# Autodesk Inventor assembly: joint4
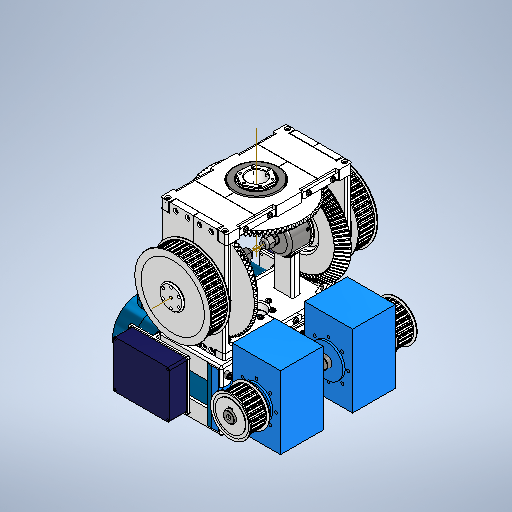
[picture p0: Inventor's stored thumbnail of the model, 512x512]
Saved by Autodesk Inventor 2025.3 (Build 293356030, 356C)
## iProperties
Created: 2025-08-31
Part Number: joint4
Document SubType Name: Assembly
Designer: MSI
Mass: 18202.1 g
Surface Area: 12604.1 cm^2
Volume: 7569.59 cm^3
Density: 2.40463 g/cm^3
Author: MSI
## Documents named in this file (32)
- C:\Users\MSI\Desktop\Project\3. 로봇팔\Robot Arm Model\joint4\joint4.iam
- C:\Users\MSI\Desktop\Project\3. 로봇팔\Robot Arm Model\joint4\encoder.ipt
- C:\Users\MSI\Desktop\Project\3. 로봇팔\Robot Arm Model\joint4\encoder_supporter.ipt
- C:\Users\MSI\Desktop\Project\3. 로봇팔\Robot Arm Model\motor1\motor.iam
- C:\Users\MSI\Desktop\Project\3. 로봇팔\Robot Arm Model\joint4\C-E6704ZZ_Autodesk_Inventor_2024_20250921\C-E6704ZZ.ipt
- C:\Users\MSI\Desktop\Project\3. 로봇팔\Robot Arm Model\joint4\C-E6810ZZ_Autodesk_Inventor_2024_20250921\C-E6810ZZ.ipt
- C:\Users\MSI\Desktop\Project\3. 로봇팔\Robot Arm Model\joint4\NTN_GS81110OuterRings\GS81110Outer Rings.ipt
- C:\Users\MSI\Desktop\Project\3. 로봇팔\Robot Arm Model\joint4\joint4\디자인 액셀러레이터\베벨 기어1.iam
- C:\Users\MSI\Desktop\Project\3. 로봇팔\Robot Arm Model\joint4\joint4\디자인 액셀러레이터\베벨 기어11.ipt
- C:\Users\MSI\Desktop\Project\3. 로봇팔\Robot Arm Model\joint4\joint4_belt_pully2\driven_pulley.iam
- C:\Users\MSI\Desktop\Project\3. 로봇팔\Robot Arm Model\joint4\joint4_belt_pully1\driving_pulley.iam
- C:\Users\MSI\Desktop\Project\3. 로봇팔\Robot Arm Model\joint4\joint4_axis2.ipt
- C:\Users\MSI\Desktop\Project\3. 로봇팔\Robot Arm Model\joint4\joint4_axis3.ipt
- C:\Users\MSI\Desktop\Project\3. 로봇팔\Robot Arm Model\joint4\joint4_pully_cover.ipt
- C:\Users\MSI\Desktop\Project\3. 로봇팔\Robot Arm Model\joint4\joint4_base.ipt
- C:\Users\MSI\Desktop\Project\3. 로봇팔\Robot Arm Model\joint4\joint4_base_carbon.ipt
- C:\Users\MSI\Desktop\Project\3. 로봇팔\Robot Arm Model\joint4\joint4_base_fixture.ipt
- C:\Users\MSI\Desktop\Project\3. 로봇팔\Robot Arm Model\joint4\joint4_base_support_1.ipt
- C:\Users\MSI\Desktop\Project\3. 로봇팔\Robot Arm Model\joint4\joint4_base_support_2.ipt
- C:\Users\MSI\Desktop\Project\3. 로봇팔\Robot Arm Model\joint4\joint4_base_support_fixture.ipt
- C:\Users\MSI\Desktop\Project\3. 로봇팔\Robot Arm Model\joint4\joint4_frame_1.ipt
- C:\Users\MSI\Desktop\Project\3. 로봇팔\Robot Arm Model\joint4\joint4_frame_2.ipt
- C:\Users\MSI\Desktop\Project\3. 로봇팔\Robot Arm Model\joint4\joint4_frame_support_1.ipt
- C:\Users\MSI\Desktop\Project\3. 로봇팔\Robot Arm Model\joint4\joint4_frame_support_2.ipt
- C:\Users\MSI\Desktop\Project\3. 로봇팔\Robot Arm Model\joint4\joint4_frame_support_fixture.ipt
- C:\Users\MSI\Desktop\Project\3. 로봇팔\Robot Arm Model\joint4\joint4_axis2_washer.ipt
- C:\Users\MSI\Desktop\Project\3. 로봇팔\Robot Arm Model\joint4\joint4_axis3_washer.ipt
- C:\Users\MSI\Desktop\Project\3. 로봇팔\Robot Arm Model\joint4\joint4_axis3_washer_2.ipt
- C:\Users\MSI\Documents\Inventor\Content Center Files\R2025\ko-KR\KS B 1023  H (2)\KS B 1023 - A  M 4 x 16 - H(1).ipt
- C:\Users\MSI\Documents\Inventor\Content Center Files\R2025\ko-KR\KS B 1023  H (2)\KS B 1023 - A  M 4 x 25 - H(1).ipt
- C:\Users\MSI\Documents\Inventor\Content Center Files\R2025\ko-KR\KS B 1012  S1\KS B 1012 - A M4(2).ipt
- C:\Users\MSI\Desktop\Project\3. 로봇팔\Robot Arm Model\Robot_Arm_Parameter.xlsx
## Components (176 placed, 30 different names)
1. motor:1 [sub-assembly] — 삽입:8, 삽입:10, 메이트:13, 메이트:14, 각도:1, 메이트:32, 메이트:33, 메이트:34, 메이트:127
2. C-E6704ZZ:1 — 삽입:6, 삽입:31
3. C-E6704ZZ:2 — 삽입:5, 삽입:30
4. C-E6810ZZ:1 — 삽입:32, 삽입:33
5. GS81110Outer Rings:1 — 삽입:13
6. GS81110Outer Rings:2 — 삽입:12, 삽입:34
7. 베벨 기어:1 [sub-assembly] — 메이트:6, 메이트:7, 삽입:11, 삽입:17, 메이트:10, 메이트:45, 메이트:46, 삽입:41, 삽입:42, 삽입:43, 삽입:44, 삽입:45, 삽입:46
8. 베벨 기어1:3 — 메이트:6, 메이트:8, 삽입:9, 메이트:47
9. joint4_axis2:1 — 삽입:9, 메이트:9, 삽입:18
10. joint4_axis2_washer:1 — 삽입:30
11. driven_pulley:1 [sub-assembly] — 삽입:15
12. driving_pulley:1 [sub-assembly] — 삽입:8
13. joint4_pully_cover:1 — 삽입:18, 삽입:15, 삽입:99, 삽입:100, 삽입:101, 삽입:102, 삽입:103, 삽입:104, 삽입:105
14. joint4_axis2:2 — 삽입:11, 삽입:21
15. joint4_axis2_washer:2 — 삽입:31
16. driven_pulley:2 [sub-assembly] — 삽입:16
17. driving_pulley:2 [sub-assembly] — 삽입:10
18. joint4_pully_cover:2 — 삽입:21, 삽입:16, 삽입:106, 삽입:107, 삽입:108, 삽입:109, 삽입:110, 삽입:111, 삽입:112
19. joint4_axis3:1 — 삽입:17, 메이트:10, 삽입:113, 각도:2, 삽입:114, 각도:3, 삽입:115, 각도:4, 삽입:116, 각도:5, 삽입:117, 각도:6, 삽입:118, 각도:7, 삽입:119, 각도:8, 삽입:120, 각도:9, 삽입:121, 각도:10, 삽입:122, 각도:11, 삽입:123, 각도:12, 삽입:124, 각도:13
20. joint4_axis3_washer:1 — 삽입:32, 삽입:14
21. joint4_axis3_washer:2 — 삽입:33
22. joint4_base:1 — 메이트:15, 메이트:16, 메이트:17, 메이트:18, 메이트:19, 메이트:20, 메이트:21, 메이트:22, 메이트:23, 메이트:27, 메이트:29, 메이트:30, 메이트:32, 메이트:33, 메이트:39, 메이트:40, 메이트:41, 메이트:56, 메이트:57, 메이트:58, 삽입:35, 삽입:36, 삽입:40, 삽입:59, 삽입:60, 삽입:61, 삽입:62, 삽입:71, 삽입:72, 삽입:73, 삽입:74
23. joint4_base:2 — 메이트:23, 메이트:24, 메이트:25, 메이트:26, 메이트:28, 메이트:31, 메이트:34, 메이트:42, 메이트:43, 메이트:44, 메이트:45, 메이트:59, 메이트:60, 삽입:37, 삽입:38, 삽입:39, 삽입:63, 삽입:64, 삽입:65, 삽입:66, 삽입:67, 삽입:68, 삽입:69, 삽입:70
24. joint4_base_support_1:1 — 메이트:48, 메이트:49, 메이트:51, 삽입:19, 메이트:56, 메이트:79, 메이트:80, 메이트:81, 메이트:82, 메이트:83, 메이트:84, 메이트:85, 메이트:86, 삽입:51, 삽입:52
25. joint4_base_support_2:1 — 메이트:48, 메이트:49, 메이트:50, 메이트:57, 메이트:58, 삽입:53, 삽입:54
26. joint4_base_carbon:5 — 메이트:79, 메이트:80
27. joint4_base_carbon:6 — 메이트:81, 메이트:82
28. joint4_base_carbon:7 — 메이트:83, 메이트:84
29. joint4_base_carbon:8 — 메이트:85, 메이트:86
30. joint4_base_support_fixture:1 — 메이트:50, 메이트:51, 삽입:75, 삽입:76
31. joint4_base_support_1:2 — 메이트:60, 삽입:55, 삽입:56
32. joint4_base_support_2:2 — 삽입:20, 메이트:59, 메이트:87, 메이트:88, 메이트:89, 메이트:90, 메이트:91, 메이트:92, 메이트:93, 메이트:94, 삽입:57, 삽입:58
33. joint4_base_carbon:9 — 메이트:87, 메이트:88
34. joint4_base_carbon:10 — 메이트:89, 메이트:90
35. joint4_base_carbon:11 — 메이트:91, 메이트:92
36. joint4_base_carbon:12 — 메이트:93, 메이트:94
37. joint4_base_support_fixture:2 — 삽입:77, 삽입:78
38. joint4_base_carbon:1 — 메이트:15, 메이트:16, 메이트:24
39. joint4_base_carbon:2 — 메이트:17, 메이트:18
40. joint4_base_carbon:3 — 메이트:19, 메이트:20
41. joint4_base_carbon:4 — 메이트:21, 메이트:22, 메이트:25
42. joint4_base_fixture:1 — 메이트:29, 메이트:30, 메이트:31, 삽입:49, 삽입:50
43. joint4_base_fixture:2 — 메이트:26, 메이트:27, 메이트:28, 삽입:47, 삽입:48
44. encoder_supporter:1 — 삽입:4, 메이트:42, 메이트:43, 메이트:44
45. encoder_supporter:2 — 삽입:7, 메이트:39, 메이트:40, 메이트:41
46. encoder:1 — 삽입:7, 메이트:47
47. encoder:2 — 삽입:4, 메이트:46
48. C-E6704ZZ:3 — 삽입:19
49. C-E6704ZZ:4 — 삽입:20
50. joint4_frame_1:1 — 메이트:63, 메이트:64, 삽입:27, 삽입:29, 메이트:75, 메이트:76, 메이트:78, 삽입:91, 삽입:92, 메이트:134
51. joint4_base_carbon:13 — 메이트:95, 메이트:96
52. joint4_base_carbon:14 — 메이트:97, 메이트:98
53. joint4_base_carbon:15 — 메이트:99, 메이트:100
54. joint4_base_carbon:16 — 메이트:101, 메이트:102
55. joint4_frame_1:2 — 메이트:61, 메이트:62, 삽입:23, 삽입:24, 메이트:73, 메이트:74, 메이트:77, 삽입:97, 삽입:98
56. joint4_base_carbon:17 — 메이트:103, 메이트:104
57. joint4_base_carbon:18 — 메이트:105, 메이트:106
58. joint4_base_carbon:19 — 메이트:107, 메이트:108
59. joint4_base_carbon:20 — 메이트:109, 메이트:110
60. joint4_frame_2:1 — 메이트:61, 메이트:62, 삽입:22, 메이트:64, 삽입:28, 메이트:7, 삽입:12, 삽입:13, 삽입:14, 메이트:77, 메이트:78, 메이트:95, 메이트:96, 메이트:97, 메이트:98, 메이트:99, 메이트:101, 메이트:103, 메이트:105, 메이트:107, 메이트:108, 메이트:109, 메이트:110, 메이트:133
61. joint4_frame_2:2 — 메이트:129, 메이트:130, 메이트:131, 메이트:132, 메이트:133, 메이트:134, 삽입:25, 메이트:63, 메이트:102, 메이트:100, 메이트:104, 메이트:106, 삽입:26
62. joint4_base_carbon:29 — 메이트:129, 메이트:130
63. joint4_base_carbon:30 — 메이트:131, 메이트:132
64. joint4_base_fixture:3 — 삽입:22, 삽입:23, 삽입:85, 삽입:86
65. joint4_base_fixture:4 — 삽입:24, 삽입:81, 삽입:82, 삽입:26
66. joint4_base_fixture:6 — 삽입:27, 삽입:79, 삽입:80, 삽입:25
67. joint4_base_fixture:5 — 삽입:28, 삽입:29, 삽입:83, 삽입:84
68. joint4_frame_support_1:1 — 메이트:65, 메이트:66, 메이트:67, 메이트:73, 삽입:6, 메이트:8, 메이트:9, 삽입:93, 삽입:94
69. joint4_base_carbon:25 — 메이트:119, 메이트:120
70. joint4_base_carbon:26 — 메이트:121, 메이트:122
71. joint4_base_carbon:27 — 메이트:123, 메이트:124
72. joint4_base_carbon:28 — 메이트:125, 메이트:126
73. joint4_frame_support_2:1 — 메이트:65, 메이트:66, 메이트:68, 메이트:74, 메이트:119, 메이트:120, 메이트:121, 메이트:122, 메이트:123, 메이트:124, 메이트:125, 메이트:126, 삽입:95, 삽입:96
74. joint4_frame_support_fixture:1 — 메이트:67, 메이트:68, 삽입:127, 삽입:128
75. joint4_frame_support_1:2 — 메이트:75, 메이트:111, 메이트:112, 메이트:113, 메이트:114, 메이트:115, 메이트:116, 메이트:117, 메이트:118, 삽입:87, 삽입:88
76. joint4_base_carbon:21 — 메이트:111, 메이트:112
77. joint4_base_carbon:22 — 메이트:113, 메이트:114
78. joint4_base_carbon:23 — 메이트:115, 메이트:116
79. joint4_base_carbon:24 — 메이트:117, 메이트:118
80. joint4_frame_support_2:2 — 메이트:76, 삽입:5, 삽입:89, 삽입:90
81. joint4_frame_support_fixture:2 — 삽입:125, 삽입:126
82. joint4_axis3_washer_2:1 — 삽입:34
83. KS B 1023 H - 미터 A  M 4 x 16 - H:1 — 삽입:47
84. KS B 1023 H - 미터 A  M 4 x 25 - H:1 — 삽입:36
85. KS B 1012 스타일 1 - 미터 A M4:1 — 삽입:113, 각도:2
86. KS B 1023 H - 미터 A  M 4 x 25 - H:2 — 삽입:35
87. KS B 1023 H - 미터 A  M 4 x 25 - H:3 — 삽입:40
88. KS B 1023 H - 미터 A  M 4 x 25 - H:4 — 삽입:38
89. KS B 1023 H - 미터 A  M 4 x 25 - H:5 — 삽입:39
90. KS B 1023 H - 미터 A  M 4 x 25 - H:6 — 삽입:37
91. KS B 1023 H - 미터 A  M 4 x 25 - H:7 — 삽입:41
92. KS B 1023 H - 미터 A  M 4 x 25 - H:8 — 삽입:46
93. KS B 1023 H - 미터 A  M 4 x 25 - H:9 — 삽입:45
94. KS B 1023 H - 미터 A  M 4 x 25 - H:10 — 삽입:43
95. KS B 1023 H - 미터 A  M 4 x 25 - H:11 — 삽입:44
96. KS B 1023 H - 미터 A  M 4 x 25 - H:12 — 삽입:42
97. KS B 1023 H - 미터 A  M 4 x 16 - H:2 — 삽입:48
98. KS B 1023 H - 미터 A  M 4 x 16 - H:3 — 삽입:49
99. KS B 1023 H - 미터 A  M 4 x 16 - H:4 — 삽입:50
100. KS B 1023 H - 미터 A  M 4 x 16 - H:5 — 삽입:52
101. KS B 1023 H - 미터 A  M 4 x 16 - H:6 — 삽입:53
102. KS B 1023 H - 미터 A  M 4 x 16 - H:7 — 삽입:54
103. KS B 1023 H - 미터 A  M 4 x 16 - H:8 — 삽입:51
104. KS B 1023 H - 미터 A  M 4 x 16 - H:9 — 삽입:56
105. KS B 1023 H - 미터 A  M 4 x 16 - H:10 — 삽입:57
106. KS B 1023 H - 미터 A  M 4 x 16 - H:11 — 삽입:55
107. KS B 1023 H - 미터 A  M 4 x 16 - H:12 — 삽입:58
108. KS B 1023 H - 미터 A  M 4 x 16 - H:13 — 삽입:60
109. KS B 1023 H - 미터 A  M 4 x 16 - H:14 — 삽입:59
110. KS B 1023 H - 미터 A  M 4 x 16 - H:15 — 삽입:62
111. KS B 1023 H - 미터 A  M 4 x 16 - H:16 — 삽입:61
112. KS B 1023 H - 미터 A  M 4 x 16 - H:17 — 삽입:64
113. KS B 1023 H - 미터 A  M 4 x 16 - H:18 — 삽입:63
114. KS B 1023 H - 미터 A  M 4 x 16 - H:19 — 삽입:65
115. KS B 1023 H - 미터 A  M 4 x 16 - H:20 — 삽입:66
116. KS B 1023 H - 미터 A  M 4 x 16 - H:21 — 삽입:72
117. KS B 1023 H - 미터 A  M 4 x 16 - H:22 — 삽입:71
118. KS B 1023 H - 미터 A  M 4 x 16 - H:23 — 삽입:74
119. KS B 1023 H - 미터 A  M 4 x 16 - H:24 — 삽입:73
120. KS B 1023 H - 미터 A  M 4 x 16 - H:25 — 삽입:67
121. KS B 1023 H - 미터 A  M 4 x 16 - H:26 — 삽입:68
122. KS B 1023 H - 미터 A  M 4 x 16 - H:27 — 삽입:70
123. KS B 1023 H - 미터 A  M 4 x 16 - H:28 — 삽입:69
124. KS B 1023 H - 미터 A  M 4 x 16 - H:29 — 삽입:76
125. KS B 1023 H - 미터 A  M 4 x 16 - H:30 — 삽입:75
126. KS B 1023 H - 미터 A  M 4 x 16 - H:31 — 삽입:78
127. KS B 1023 H - 미터 A  M 4 x 16 - H:32 — 삽입:77
128. KS B 1023 H - 미터 A  M 4 x 16 - H:33 — 삽입:88
129. KS B 1023 H - 미터 A  M 4 x 16 - H:34 — 삽입:89
130. KS B 1023 H - 미터 A  M 4 x 16 - H:35 — 삽입:90
131. KS B 1023 H - 미터 A  M 4 x 16 - H:36 — 삽입:87
132. KS B 1023 H - 미터 A  M 4 x 16 - H:37 — 삽입:94
133. KS B 1023 H - 미터 A  M 4 x 16 - H:38 — 삽입:95
134. KS B 1023 H - 미터 A  M 4 x 16 - H:39 — 삽입:93
135. KS B 1023 H - 미터 A  M 4 x 16 - H:40 — 삽입:96
136. KS B 1023 H - 미터 A  M 4 x 16 - H:41 — 삽입:91
137. KS B 1023 H - 미터 A  M 4 x 16 - H:42 — 삽입:92
138. KS B 1023 H - 미터 A  M 4 x 16 - H:43 — 삽입:98
139. KS B 1023 H - 미터 A  M 4 x 16 - H:44 — 삽입:97
140. KS B 1023 H - 미터 A  M 4 x 16 - H:45 — 삽입:79
141. KS B 1023 H - 미터 A  M 4 x 16 - H:46 — 삽입:80
142. KS B 1023 H - 미터 A  M 4 x 16 - H:47 — 삽입:83
143. KS B 1023 H - 미터 A  M 4 x 16 - H:48 — 삽입:84
144. KS B 1023 H - 미터 A  M 4 x 16 - H:49 — 삽입:81
145. KS B 1023 H - 미터 A  M 4 x 16 - H:50 — 삽입:82
146. KS B 1023 H - 미터 A  M 4 x 16 - H:51 — 삽입:85
147. KS B 1023 H - 미터 A  M 4 x 16 - H:52 — 삽입:86
148. KS B 1023 H - 미터 A  M 4 x 16 - H:53 — 삽입:100
149. KS B 1023 H - 미터 A  M 4 x 16 - H:54 — 삽입:101
150. KS B 1023 H - 미터 A  M 4 x 16 - H:55 — 삽입:102
151. KS B 1023 H - 미터 A  M 4 x 16 - H:56 — 삽입:103
152. KS B 1023 H - 미터 A  M 4 x 16 - H:57 — 삽입:104
153. KS B 1023 H - 미터 A  M 4 x 16 - H:58 — 삽입:105
154. KS B 1023 H - 미터 A  M 4 x 16 - H:59 — 삽입:99
155. KS B 1023 H - 미터 A  M 4 x 16 - H:60 — 삽입:107
156. KS B 1023 H - 미터 A  M 4 x 16 - H:61 — 삽입:108
157. KS B 1023 H - 미터 A  M 4 x 16 - H:62 — 삽입:109
158. KS B 1023 H - 미터 A  M 4 x 16 - H:63 — 삽입:110
159. KS B 1023 H - 미터 A  M 4 x 16 - H:64 — 삽입:111
160. KS B 1023 H - 미터 A  M 4 x 16 - H:65 — 삽입:112
161. KS B 1023 H - 미터 A  M 4 x 16 - H:66 — 삽입:106
162. KS B 1012 스타일 1 - 미터 A M4:2 — 삽입:114, 각도:3
163. KS B 1012 스타일 1 - 미터 A M4:3 — 삽입:115, 각도:4
164. KS B 1012 스타일 1 - 미터 A M4:4 — 삽입:116, 각도:5
165. KS B 1012 스타일 1 - 미터 A M4:5 — 삽입:117, 각도:6
166. KS B 1012 스타일 1 - 미터 A M4:6 — 삽입:118, 각도:7
167. KS B 1012 스타일 1 - 미터 A M4:7 — 삽입:120, 각도:9
168. KS B 1012 스타일 1 - 미터 A M4:8 — 삽입:119, 각도:8
169. KS B 1012 스타일 1 - 미터 A M4:9 — 삽입:121, 각도:10
170. KS B 1012 스타일 1 - 미터 A M4:10 — 삽입:122, 각도:11
171. KS B 1012 스타일 1 - 미터 A M4:11 — 삽입:123, 각도:12
172. KS B 1012 스타일 1 - 미터 A M4:12 — 삽입:124, 각도:13
173. KS B 1023 H - 미터 A  M 4 x 16 - H:67 — 삽입:125
174. KS B 1023 H - 미터 A  M 4 x 16 - H:68 — 삽입:126
175. KS B 1023 H - 미터 A  M 4 x 16 - H:69 — 삽입:127
176. KS B 1023 H - 미터 A  M 4 x 16 - H:70 — 삽입:128
## Relationships (260: Insert 125, Mate 122, Angle 13)
- 삽입:4 [Insert]: encoder_supporter:1 ↔ encoder:2
- 삽입:5 [Insert]: C-E6704ZZ:2 ↔ joint4_frame_support_2:2
- 삽입:6 [Insert]: C-E6704ZZ:1 ↔ joint4_frame_support_1:1
- 메이트:6 [Mate]: 베벨 기어:1 ↔ 베벨 기어1:3
- 삽입:7 [Insert]: encoder_supporter:2 ↔ encoder:1
- 메이트:7 [Mate]: 베벨 기어:1 ↔ joint4_frame_2:1
- 메이트:8 [Mate]: 베벨 기어1:3 ↔ joint4_frame_support_1:1
- 삽입:8 [Insert]: motor:1 ↔ driving_pulley:1
- 삽입:9 [Insert]: 베벨 기어1:3 ↔ joint4_axis2:1
- 삽입:10 [Insert]: motor:1 ↔ driving_pulley:2
- 삽입:11 [Insert]: 베벨 기어:1 ↔ joint4_axis2:2
- 삽입:12 [Insert]: GS81110Outer Rings:2 ↔ joint4_frame_2:1
- 삽입:13 [Insert]: GS81110Outer Rings:1 ↔ joint4_frame_2:1
- 삽입:14 [Insert] (0.25 mm): joint4_axis3_washer:1 ↔ joint4_frame_2:1
- 메이트:9 [Mate]: joint4_axis2:1 ↔ joint4_frame_support_1:1
- 삽입:15 [Insert]: driven_pulley:1 ↔ joint4_pully_cover:1
- 삽입:16 [Insert]: driven_pulley:2 ↔ joint4_pully_cover:2
- 삽입:17 [Insert]: 베벨 기어:1 ↔ joint4_axis3:1
- 메이트:10 [Mate]: 베벨 기어:1 ↔ joint4_axis3:1
- 삽입:18 [Insert] (0.5 mm): joint4_axis2:1 ↔ joint4_pully_cover:1
- 메이트:13 [Mate]: motor:1
- 메이트:14 [Mate]: motor:1
- 각도:1 [Angle] (0 deg): motor:1
- 메이트:15 [Mate]: joint4_base:1 ↔ joint4_base_carbon:1
- 메이트:16 [Mate]: joint4_base:1 ↔ joint4_base_carbon:1
- 메이트:17 [Mate]: joint4_base:1 ↔ joint4_base_carbon:2
- 메이트:18 [Mate]: joint4_base:1 ↔ joint4_base_carbon:2
- 메이트:19 [Mate]: joint4_base:1 ↔ joint4_base_carbon:3
- 메이트:20 [Mate]: joint4_base:1 ↔ joint4_base_carbon:3
- 메이트:21 [Mate]: joint4_base:1 ↔ joint4_base_carbon:4
- 메이트:22 [Mate]: joint4_base:1 ↔ joint4_base_carbon:4
- 메이트:23 [Mate]: joint4_base:1 ↔ joint4_base:2
- 메이트:24 [Mate]: joint4_base:2 ↔ joint4_base_carbon:1
- 메이트:25 [Mate]: joint4_base:2 ↔ joint4_base_carbon:4
- 메이트:26 [Mate]: joint4_base:2 ↔ joint4_base_fixture:2
- 메이트:27 [Mate]: joint4_base:1 ↔ joint4_base_fixture:2
- 메이트:28 [Mate]: joint4_base:2 ↔ joint4_base_fixture:2
- 메이트:29 [Mate]: joint4_base:1 ↔ joint4_base_fixture:1
- 메이트:30 [Mate]: joint4_base:1 ↔ joint4_base_fixture:1
- 메이트:31 [Mate]: joint4_base:2 ↔ joint4_base_fixture:1
- 메이트:32 [Mate]: motor:1 ↔ joint4_base:1
- 메이트:33 [Mate]: motor:1 ↔ joint4_base:1
- 메이트:34 [Mate]: motor:1 ↔ joint4_base:2
- 메이트:39 [Mate]: joint4_base:1 ↔ encoder_supporter:2
- 메이트:40 [Mate]: joint4_base:1 ↔ encoder_supporter:2
- 메이트:41 [Mate]: joint4_base:1 ↔ encoder_supporter:2
- 메이트:42 [Mate]: joint4_base:2 ↔ encoder_supporter:1
- 메이트:43 [Mate]: joint4_base:2 ↔ encoder_supporter:1
- 메이트:44 [Mate]: joint4_base:2 ↔ encoder_supporter:1
- 메이트:45 [Mate]: 베벨 기어:1 ↔ joint4_base:2
- 메이트:46 [Mate]: 베벨 기어:1 ↔ encoder:2
- 메이트:47 [Mate]: 베벨 기어1:3 ↔ encoder:1
- 메이트:48 [Mate]: joint4_base_support_1:1 ↔ joint4_base_support_2:1
- 메이트:49 [Mate]: joint4_base_support_1:1 ↔ joint4_base_support_2:1
- 메이트:50 [Mate]: joint4_base_support_2:1 ↔ joint4_base_support_fixture:1
- 메이트:51 [Mate]: joint4_base_support_1:1 ↔ joint4_base_support_fixture:1
- [Mate]: joint4_base_support_1:2 ↔ joint4_base_support_2:2
- [Mate]: joint4_base_support_1:2 ↔ joint4_base_support_2:2
- [Mate]: joint4_base_support_2:2 ↔ joint4_base_support_fixture:2
- [Mate]: joint4_base_support_1:2 ↔ joint4_base_support_fixture:2
- 삽입:19 [Insert]: joint4_base_support_1:1 ↔ C-E6704ZZ:3
- 메이트:56 [Mate]: joint4_base:1 ↔ joint4_base_support_1:1
- 메이트:57 [Mate]: joint4_base:1 ↔ joint4_base_support_2:1
- 메이트:58 [Mate]: joint4_base:1 ↔ joint4_base_support_2:1
- 삽입:20 [Insert]: joint4_base_support_2:2 ↔ C-E6704ZZ:4
- 메이트:59 [Mate]: joint4_base:2 ↔ joint4_base_support_2:2
- 메이트:60 [Mate]: joint4_base:2 ↔ joint4_base_support_1:2
- 삽입:21 [Insert] (0.5 mm): joint4_axis2:2 ↔ joint4_pully_cover:2
- 메이트:61 [Mate]: joint4_frame_1:2 ↔ joint4_frame_2:1
- 메이트:62 [Mate]: joint4_frame_1:2 ↔ joint4_frame_2:1
- 삽입:22 [Insert]: joint4_frame_2:1 ↔ joint4_base_fixture:3
- 삽입:23 [Insert]: joint4_frame_1:2 ↔ joint4_base_fixture:3
- 삽입:24 [Insert]: joint4_frame_1:2 ↔ joint4_base_fixture:4
- 삽입:25 [Insert]: joint4_frame_2:2 ↔ joint4_base_fixture:6
- 메이트:63 [Mate]: joint4_frame_1:1 ↔ joint4_frame_2:2
- 메이트:64 [Mate]: joint4_frame_1:1 ↔ joint4_frame_2:1
- 삽입:26 [Insert]: joint4_frame_2:2 ↔ joint4_base_fixture:4
- 삽입:27 [Insert]: joint4_frame_1:1 ↔ joint4_base_fixture:6
- 삽입:28 [Insert]: joint4_frame_2:1 ↔ joint4_base_fixture:5
- 삽입:29 [Insert]: joint4_frame_1:1 ↔ joint4_base_fixture:5
- 메이트:65 [Mate]: joint4_frame_support_1:1 ↔ joint4_frame_support_2:1
- 메이트:66 [Mate]: joint4_frame_support_1:1 ↔ joint4_frame_support_2:1
- 메이트:67 [Mate]: joint4_frame_support_1:1 ↔ joint4_frame_support_fixture:1
- 메이트:68 [Mate]: joint4_frame_support_2:1 ↔ joint4_frame_support_fixture:1
- [Mate]: joint4_frame_support_1:2 ↔ joint4_frame_support_2:2
- [Mate]: joint4_frame_support_1:2 ↔ joint4_frame_support_2:2
- [Mate]: joint4_frame_support_1:2 ↔ joint4_frame_support_fixture:2
- [Mate]: joint4_frame_support_2:2 ↔ joint4_frame_support_fixture:2
- 메이트:73 [Mate]: joint4_frame_1:2 ↔ joint4_frame_support_1:1
- 메이트:74 [Mate]: joint4_frame_1:2 ↔ joint4_frame_support_2:1
- 메이트:75 [Mate]: joint4_frame_1:1 ↔ joint4_frame_support_1:2
- 메이트:76 [Mate]: joint4_frame_1:1 ↔ joint4_frame_support_2:2
- 메이트:77 [Mate] (0.5 mm): joint4_frame_1:2 ↔ joint4_frame_2:1
- 메이트:78 [Mate] (0.5 mm): joint4_frame_1:1 ↔ joint4_frame_2:1
- 메이트:79 [Mate] (0.25 mm): joint4_base_support_1:1 ↔ joint4_base_carbon:5
- 메이트:80 [Mate]: joint4_base_support_1:1 ↔ joint4_base_carbon:5
- 메이트:81 [Mate] (0.25 mm): joint4_base_support_1:1 ↔ joint4_base_carbon:6
- 메이트:82 [Mate]: joint4_base_support_1:1 ↔ joint4_base_carbon:6
- 메이트:83 [Mate] (0.25 mm): joint4_base_support_1:1 ↔ joint4_base_carbon:7
- 메이트:84 [Mate]: joint4_base_support_1:1 ↔ joint4_base_carbon:7
- 메이트:85 [Mate] (0.25 mm): joint4_base_support_1:1 ↔ joint4_base_carbon:8
- 메이트:86 [Mate]: joint4_base_support_1:1 ↔ joint4_base_carbon:8
- 메이트:87 [Mate] (0.25 mm): joint4_base_support_2:2 ↔ joint4_base_carbon:9
- 메이트:88 [Mate]: joint4_base_support_2:2 ↔ joint4_base_carbon:9
- 메이트:89 [Mate] (0.25 mm): joint4_base_support_2:2 ↔ joint4_base_carbon:10
- 메이트:90 [Mate]: joint4_base_support_2:2 ↔ joint4_base_carbon:10
- 메이트:91 [Mate] (0.25 mm): joint4_base_support_2:2 ↔ joint4_base_carbon:11
- 메이트:92 [Mate]: joint4_base_support_2:2 ↔ joint4_base_carbon:11
- 메이트:93 [Mate] (0.25 mm): joint4_base_support_2:2 ↔ joint4_base_carbon:12
- 메이트:94 [Mate]: joint4_base_support_2:2 ↔ joint4_base_carbon:12
- 메이트:95 [Mate] (0.25 mm): joint4_base_carbon:13 ↔ joint4_frame_2:1
- 메이트:96 [Mate]: joint4_base_carbon:13 ↔ joint4_frame_2:1
- 메이트:97 [Mate] (0.25 mm): joint4_base_carbon:14 ↔ joint4_frame_2:1
- 메이트:98 [Mate]: joint4_base_carbon:14 ↔ joint4_frame_2:1
- 메이트:99 [Mate] (0.25 mm): joint4_base_carbon:15 ↔ joint4_frame_2:1
- 메이트:100 [Mate]: joint4_base_carbon:15 ↔ joint4_frame_2:2
- 메이트:101 [Mate] (0.25 mm): joint4_base_carbon:16 ↔ joint4_frame_2:1
- 메이트:102 [Mate]: joint4_base_carbon:16 ↔ joint4_frame_2:2
- 메이트:103 [Mate] (0.25 mm): joint4_base_carbon:17 ↔ joint4_frame_2:1
- 메이트:104 [Mate]: joint4_base_carbon:17 ↔ joint4_frame_2:2
- 메이트:105 [Mate] (0.25 mm): joint4_base_carbon:18 ↔ joint4_frame_2:1
- 메이트:106 [Mate]: joint4_base_carbon:18 ↔ joint4_frame_2:2
- 메이트:107 [Mate] (0.25 mm): joint4_base_carbon:19 ↔ joint4_frame_2:1
- 메이트:108 [Mate]: joint4_base_carbon:19 ↔ joint4_frame_2:1
- 메이트:109 [Mate] (0.25 mm): joint4_base_carbon:20 ↔ joint4_frame_2:1
- 메이트:110 [Mate]: joint4_base_carbon:20 ↔ joint4_frame_2:1
- 메이트:111 [Mate] (0.25 mm): joint4_frame_support_1:2 ↔ joint4_base_carbon:21
- 메이트:112 [Mate]: joint4_frame_support_1:2 ↔ joint4_base_carbon:21
- 메이트:113 [Mate] (0.25 mm): joint4_frame_support_1:2 ↔ joint4_base_carbon:22
- 메이트:114 [Mate]: joint4_frame_support_1:2 ↔ joint4_base_carbon:22
- 메이트:115 [Mate] (0.25 mm): joint4_frame_support_1:2 ↔ joint4_base_carbon:23
- 메이트:116 [Mate]: joint4_frame_support_1:2 ↔ joint4_base_carbon:23
- 메이트:117 [Mate] (0.25 mm): joint4_frame_support_1:2 ↔ joint4_base_carbon:24
- 메이트:118 [Mate]: joint4_frame_support_1:2 ↔ joint4_base_carbon:24
- 메이트:119 [Mate] (0.25 mm): joint4_base_carbon:25 ↔ joint4_frame_support_2:1
- 메이트:120 [Mate]: joint4_base_carbon:25 ↔ joint4_frame_support_2:1
- 메이트:121 [Mate] (0.25 mm): joint4_base_carbon:26 ↔ joint4_frame_support_2:1
- 메이트:122 [Mate]: joint4_base_carbon:26 ↔ joint4_frame_support_2:1
- 메이트:123 [Mate] (0.25 mm): joint4_base_carbon:27 ↔ joint4_frame_support_2:1
- 메이트:124 [Mate]: joint4_base_carbon:27 ↔ joint4_frame_support_2:1
- 메이트:125 [Mate] (0.25 mm): joint4_base_carbon:28 ↔ joint4_frame_support_2:1
- 메이트:126 [Mate]: joint4_base_carbon:28 ↔ joint4_frame_support_2:1
- 삽입:30 [Insert] (0.5 mm): C-E6704ZZ:2 ↔ joint4_axis2_washer:1
- 삽입:31 [Insert] (0.5 mm): C-E6704ZZ:1 ↔ joint4_axis2_washer:2
- 삽입:32 [Insert] (0.25 mm): C-E6810ZZ:1 ↔ joint4_axis3_washer:1
- 삽입:33 [Insert] (0.25 mm): C-E6810ZZ:1 ↔ joint4_axis3_washer:2
- 삽입:34 [Insert] (0.5 mm): GS81110Outer Rings:2 ↔ joint4_axis3_washer_2:1
- 삽입:35 [Insert]: joint4_base:1 ↔ KS B 1023 H - 미터 A  M 4 x 25 - H:2
- 삽입:36 [Insert]: joint4_base:1 ↔ KS B 1023 H - 미터 A  M 4 x 25 - H:1
- 삽입:37 [Insert]: joint4_base:2 ↔ KS B 1023 H - 미터 A  M 4 x 25 - H:6
- 삽입:38 [Insert]: joint4_base:2 ↔ KS B 1023 H - 미터 A  M 4 x 25 - H:4
- 삽입:39 [Insert]: joint4_base:2 ↔ KS B 1023 H - 미터 A  M 4 x 25 - H:5
- 삽입:40 [Insert]: joint4_base:1 ↔ KS B 1023 H - 미터 A  M 4 x 25 - H:3
- 삽입:41 [Insert]: 베벨 기어:1 ↔ KS B 1023 H - 미터 A  M 4 x 25 - H:7
- 삽입:42 [Insert]: 베벨 기어:1 ↔ KS B 1023 H - 미터 A  M 4 x 25 - H:12
- 삽입:43 [Insert]: 베벨 기어:1 ↔ KS B 1023 H - 미터 A  M 4 x 25 - H:10
- 삽입:44 [Insert]: 베벨 기어:1 ↔ KS B 1023 H - 미터 A  M 4 x 25 - H:11
- 삽입:45 [Insert]: 베벨 기어:1 ↔ KS B 1023 H - 미터 A  M 4 x 25 - H:9
- 삽입:46 [Insert]: 베벨 기어:1 ↔ KS B 1023 H - 미터 A  M 4 x 25 - H:8
- 삽입:47 [Insert]: joint4_base_fixture:2 ↔ KS B 1023 H - 미터 A  M 4 x 16 - H:1
- 삽입:48 [Insert]: joint4_base_fixture:2 ↔ KS B 1023 H - 미터 A  M 4 x 16 - H:2
- 삽입:49 [Insert]: joint4_base_fixture:1 ↔ KS B 1023 H - 미터 A  M 4 x 16 - H:3
- 삽입:50 [Insert]: joint4_base_fixture:1 ↔ KS B 1023 H - 미터 A  M 4 x 16 - H:4
- 삽입:51 [Insert]: joint4_base_support_1:1 ↔ KS B 1023 H - 미터 A  M 4 x 16 - H:8
- 삽입:52 [Insert]: joint4_base_support_1:1 ↔ KS B 1023 H - 미터 A  M 4 x 16 - H:5
- 삽입:53 [Insert]: joint4_base_support_2:1 ↔ KS B 1023 H - 미터 A  M 4 x 16 - H:6
- 삽입:54 [Insert]: joint4_base_support_2:1 ↔ KS B 1023 H - 미터 A  M 4 x 16 - H:7
- 삽입:55 [Insert]: joint4_base_support_1:2 ↔ KS B 1023 H - 미터 A  M 4 x 16 - H:11
- 삽입:56 [Insert]: joint4_base_support_1:2 ↔ KS B 1023 H - 미터 A  M 4 x 16 - H:9
- 삽입:57 [Insert]: joint4_base_support_2:2 ↔ KS B 1023 H - 미터 A  M 4 x 16 - H:10
- 삽입:58 [Insert]: joint4_base_support_2:2 ↔ KS B 1023 H - 미터 A  M 4 x 16 - H:12
- 삽입:59 [Insert]: joint4_base:1 ↔ KS B 1023 H - 미터 A  M 4 x 16 - H:14
- 삽입:60 [Insert]: joint4_base:1 ↔ KS B 1023 H - 미터 A  M 4 x 16 - H:13
- 삽입:61 [Insert]: joint4_base:1 ↔ KS B 1023 H - 미터 A  M 4 x 16 - H:16
- 삽입:62 [Insert]: joint4_base:1 ↔ KS B 1023 H - 미터 A  M 4 x 16 - H:15
- 삽입:63 [Insert]: joint4_base:2 ↔ KS B 1023 H - 미터 A  M 4 x 16 - H:18
- 삽입:64 [Insert]: joint4_base:2 ↔ KS B 1023 H - 미터 A  M 4 x 16 - H:17
- 삽입:65 [Insert]: joint4_base:2 ↔ KS B 1023 H - 미터 A  M 4 x 16 - H:19
- 삽입:66 [Insert]: joint4_base:2 ↔ KS B 1023 H - 미터 A  M 4 x 16 - H:20
- 삽입:67 [Insert]: joint4_base:2 ↔ KS B 1023 H - 미터 A  M 4 x 16 - H:25
- 삽입:68 [Insert]: joint4_base:2 ↔ KS B 1023 H - 미터 A  M 4 x 16 - H:26
- 삽입:69 [Insert]: joint4_base:2 ↔ KS B 1023 H - 미터 A  M 4 x 16 - H:28
- 삽입:70 [Insert]: joint4_base:2 ↔ KS B 1023 H - 미터 A  M 4 x 16 - H:27
- 삽입:71 [Insert]: joint4_base:1 ↔ KS B 1023 H - 미터 A  M 4 x 16 - H:22
- 삽입:72 [Insert]: joint4_base:1 ↔ KS B 1023 H - 미터 A  M 4 x 16 - H:21
- 삽입:73 [Insert]: joint4_base:1 ↔ KS B 1023 H - 미터 A  M 4 x 16 - H:24
- 삽입:74 [Insert]: joint4_base:1 ↔ KS B 1023 H - 미터 A  M 4 x 16 - H:23
- 삽입:75 [Insert]: joint4_base_support_fixture:1 ↔ KS B 1023 H - 미터 A  M 4 x 16 - H:30
- 삽입:76 [Insert]: joint4_base_support_fixture:1 ↔ KS B 1023 H - 미터 A  M 4 x 16 - H:29
- 삽입:77 [Insert]: joint4_base_support_fixture:2 ↔ KS B 1023 H - 미터 A  M 4 x 16 - H:32
- 삽입:78 [Insert]: joint4_base_support_fixture:2 ↔ KS B 1023 H - 미터 A  M 4 x 16 - H:31
- 삽입:79 [Insert]: joint4_base_fixture:6 ↔ KS B 1023 H - 미터 A  M 4 x 16 - H:45
- 삽입:80 [Insert]: joint4_base_fixture:6 ↔ KS B 1023 H - 미터 A  M 4 x 16 - H:46
- 삽입:81 [Insert]: joint4_base_fixture:4 ↔ KS B 1023 H - 미터 A  M 4 x 16 - H:49
- 삽입:82 [Insert]: joint4_base_fixture:4 ↔ KS B 1023 H - 미터 A  M 4 x 16 - H:50
- 삽입:83 [Insert]: joint4_base_fixture:5 ↔ KS B 1023 H - 미터 A  M 4 x 16 - H:47
- 삽입:84 [Insert]: joint4_base_fixture:5 ↔ KS B 1023 H - 미터 A  M 4 x 16 - H:48
- 삽입:85 [Insert]: joint4_base_fixture:3 ↔ KS B 1023 H - 미터 A  M 4 x 16 - H:51
- 삽입:86 [Insert]: joint4_base_fixture:3 ↔ KS B 1023 H - 미터 A  M 4 x 16 - H:52
- 삽입:87 [Insert]: joint4_frame_support_1:2 ↔ KS B 1023 H - 미터 A  M 4 x 16 - H:36
- 삽입:88 [Insert]: joint4_frame_support_1:2 ↔ KS B 1023 H - 미터 A  M 4 x 16 - H:33
- 삽입:89 [Insert]: joint4_frame_support_2:2 ↔ KS B 1023 H - 미터 A  M 4 x 16 - H:34
- 삽입:90 [Insert]: joint4_frame_support_2:2 ↔ KS B 1023 H - 미터 A  M 4 x 16 - H:35
- 삽입:91 [Insert]: joint4_frame_1:1 ↔ KS B 1023 H - 미터 A  M 4 x 16 - H:41
- 삽입:92 [Insert]: joint4_frame_1:1 ↔ KS B 1023 H - 미터 A  M 4 x 16 - H:42
- 삽입:93 [Insert]: joint4_frame_support_1:1 ↔ KS B 1023 H - 미터 A  M 4 x 16 - H:39
- 삽입:94 [Insert]: joint4_frame_support_1:1 ↔ KS B 1023 H - 미터 A  M 4 x 16 - H:37
- 삽입:95 [Insert]: joint4_frame_support_2:1 ↔ KS B 1023 H - 미터 A  M 4 x 16 - H:38
- 삽입:96 [Insert]: joint4_frame_support_2:1 ↔ KS B 1023 H - 미터 A  M 4 x 16 - H:40
- 삽입:97 [Insert]: joint4_frame_1:2 ↔ KS B 1023 H - 미터 A  M 4 x 16 - H:44
- 삽입:98 [Insert]: joint4_frame_1:2 ↔ KS B 1023 H - 미터 A  M 4 x 16 - H:43
- 삽입:99 [Insert]: joint4_pully_cover:1 ↔ KS B 1023 H - 미터 A  M 4 x 16 - H:59
- 삽입:100 [Insert]: joint4_pully_cover:1 ↔ KS B 1023 H - 미터 A  M 4 x 16 - H:53
- 삽입:101 [Insert]: joint4_pully_cover:1 ↔ KS B 1023 H - 미터 A  M 4 x 16 - H:54
- 삽입:102 [Insert]: joint4_pully_cover:1 ↔ KS B 1023 H - 미터 A  M 4 x 16 - H:55
- 삽입:103 [Insert]: joint4_pully_cover:1 ↔ KS B 1023 H - 미터 A  M 4 x 16 - H:56
- 삽입:104 [Insert]: joint4_pully_cover:1 ↔ KS B 1023 H - 미터 A  M 4 x 16 - H:57
- 삽입:105 [Insert]: joint4_pully_cover:1 ↔ KS B 1023 H - 미터 A  M 4 x 16 - H:58
- 삽입:106 [Insert]: joint4_pully_cover:2 ↔ KS B 1023 H - 미터 A  M 4 x 16 - H:66
- 삽입:107 [Insert]: joint4_pully_cover:2 ↔ KS B 1023 H - 미터 A  M 4 x 16 - H:60
- 삽입:108 [Insert]: joint4_pully_cover:2 ↔ KS B 1023 H - 미터 A  M 4 x 16 - H:61
- 삽입:109 [Insert]: joint4_pully_cover:2 ↔ KS B 1023 H - 미터 A  M 4 x 16 - H:62
- 삽입:110 [Insert]: joint4_pully_cover:2 ↔ KS B 1023 H - 미터 A  M 4 x 16 - H:63
- 삽입:111 [Insert]: joint4_pully_cover:2 ↔ KS B 1023 H - 미터 A  M 4 x 16 - H:64
- 삽입:112 [Insert]: joint4_pully_cover:2 ↔ KS B 1023 H - 미터 A  M 4 x 16 - H:65
- 삽입:113 [Insert]: joint4_axis3:1 ↔ KS B 1012 스타일 1 - 미터 A M4:1
- 각도:2 [Angle] (0 deg): joint4_axis3:1 ↔ KS B 1012 스타일 1 - 미터 A M4:1
- 삽입:114 [Insert]: joint4_axis3:1 ↔ KS B 1012 스타일 1 - 미터 A M4:2
- 각도:3 [Angle] (0 deg): joint4_axis3:1 ↔ KS B 1012 스타일 1 - 미터 A M4:2
- 삽입:115 [Insert]: joint4_axis3:1 ↔ KS B 1012 스타일 1 - 미터 A M4:3
- 각도:4 [Angle] (0 deg): joint4_axis3:1 ↔ KS B 1012 스타일 1 - 미터 A M4:3
- 삽입:116 [Insert]: joint4_axis3:1 ↔ KS B 1012 스타일 1 - 미터 A M4:4
- 각도:5 [Angle] (0 deg): joint4_axis3:1 ↔ KS B 1012 스타일 1 - 미터 A M4:4
- 삽입:117 [Insert]: joint4_axis3:1 ↔ KS B 1012 스타일 1 - 미터 A M4:5
- 각도:6 [Angle] (0 deg): joint4_axis3:1 ↔ KS B 1012 스타일 1 - 미터 A M4:5
- 삽입:118 [Insert]: joint4_axis3:1 ↔ KS B 1012 스타일 1 - 미터 A M4:6
- 각도:7 [Angle] (0 deg): joint4_axis3:1 ↔ KS B 1012 스타일 1 - 미터 A M4:6
- 삽입:119 [Insert]: joint4_axis3:1 ↔ KS B 1012 스타일 1 - 미터 A M4:8
- 각도:8 [Angle] (0 deg): joint4_axis3:1 ↔ KS B 1012 스타일 1 - 미터 A M4:8
- 삽입:120 [Insert]: joint4_axis3:1 ↔ KS B 1012 스타일 1 - 미터 A M4:7
- 각도:9 [Angle] (0 deg): joint4_axis3:1 ↔ KS B 1012 스타일 1 - 미터 A M4:7
- 삽입:121 [Insert]: joint4_axis3:1 ↔ KS B 1012 스타일 1 - 미터 A M4:9
- 각도:10 [Angle] (0 deg): joint4_axis3:1 ↔ KS B 1012 스타일 1 - 미터 A M4:9
- 삽입:122 [Insert]: joint4_axis3:1 ↔ KS B 1012 스타일 1 - 미터 A M4:10
- 각도:11 [Angle] (0 deg): joint4_axis3:1 ↔ KS B 1012 스타일 1 - 미터 A M4:10
- 삽입:123 [Insert]: joint4_axis3:1 ↔ KS B 1012 스타일 1 - 미터 A M4:11
- 각도:12 [Angle] (0 deg): joint4_axis3:1 ↔ KS B 1012 스타일 1 - 미터 A M4:11
- 삽입:124 [Insert]: joint4_axis3:1 ↔ KS B 1012 스타일 1 - 미터 A M4:12
- 각도:13 [Angle] (0 deg): joint4_axis3:1 ↔ KS B 1012 스타일 1 - 미터 A M4:12
- 메이트:127 [Mate]: motor:1
- 삽입:125 [Insert]: joint4_frame_support_fixture:2 ↔ KS B 1023 H - 미터 A  M 4 x 16 - H:67
- 삽입:126 [Insert]: joint4_frame_support_fixture:2 ↔ KS B 1023 H - 미터 A  M 4 x 16 - H:68
- 삽입:127 [Insert]: joint4_frame_support_fixture:1 ↔ KS B 1023 H - 미터 A  M 4 x 16 - H:69
- 삽입:128 [Insert]: joint4_frame_support_fixture:1 ↔ KS B 1023 H - 미터 A  M 4 x 16 - H:70
- 메이트:129 [Mate] (0.25 mm): joint4_frame_2:2 ↔ joint4_base_carbon:29
- 메이트:130 [Mate]: joint4_frame_2:2 ↔ joint4_base_carbon:29
- 메이트:131 [Mate] (0.25 mm): joint4_frame_2:2 ↔ joint4_base_carbon:30
- 메이트:132 [Mate]: joint4_frame_2:2 ↔ joint4_base_carbon:30
- 메이트:133 [Mate]: joint4_frame_2:1 ↔ joint4_frame_2:2
- 메이트:134 [Mate]: joint4_frame_1:1 ↔ joint4_frame_2:2
## Named parameters: joint4_belt_centor = 157.367 mm, joint4_axis2_L = 58.803 mm, joint4_axis2_b1 = 35 mm, joint4_axis2_b2 = 10 mm, joint4_axis2_d = 19 mm, joint4_miter_m = 2 mm, joint4_miter_a = 20 deg, joint4_miter_z = 79 mm, joint4_miter_b = 6.90139 mm, joint4_axis3_L = 23.5 mm, joint4_axis3_d1 = 30 mm, joint4_axis3_d2 = 50 mm, joint3_belt_centor = 157.367 mm, joint3_axis2_L = 63.75 mm, joint3_axis2_b1 = 38 mm, joint3_axis2_d = 29 mm, joint3_planetary_m = 2 mm, joint3_planetary_a = 20 deg, joint3_planetary_np = 4 mm, joint3_sun_z = 20 mm, joint3_sun_b = 19 mm, joint3_planet_z = 20 mm, joint3_planet_b = 19 mm, joint3_ring_z = 60 mm, joint3_ring_b = 18 mm, joint3_axis3_L = 20 mm, joint3_axis3_d = 29 mm, joint3_miter_m = 4 mm, joint3_miter_a = 20 deg, joint3_miter_z = 28 mm, joint3_miter_b = 25.07657 mm, joint3_axis4_L = 43.706 mm, joint3_axis4_d1 = 30 mm, joint3_axis4_d2 = 50 mm, d156_d152 = 0 mm, d157_d153 = 0 mm, d158_d154 = 0 mm, d159_d155 = 0 mm, d186_d180 = 0 mm, d187_d181 = 0 mm, d188_d184 = 0 mm, d189_d185 = 0 mm, joint3_miter_z2 = 39 mm, joint3_miter_z1 = 26 mm
